# Autodesk Inventor assembly: ASY PRS DrainSystemBottom_940
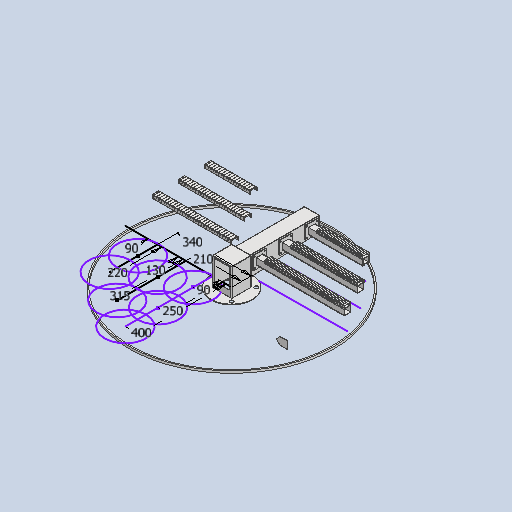
[picture p0: Inventor's stored thumbnail of the model, 512x512]
Saved by Autodesk Inventor 2026.2 (Build 302298000, 298)
## iProperties
Created: 2026-05-12
Part Number: ASY PRS DrainSystemBottom_940
Document SubType Name: Assembly
Designer: admin
Author: admin
## Documents named in this file (20)
- C:\Users\admin\Documents\Inventor\PRS-Purovsk\ASY-PRS-DRS 940.iam
- C:\Users\admin\Documents\Inventor\PRS-Purovsk\PRS-1425 FDS Way FLANGE.ipt
- C:\Users\admin\Documents\Inventor\PRS-Purovsk\ANP 1401 DSB DIMentions.ipt
- C:\Users\admin\Documents\Inventor\PRS-Purovsk\PRS-1662 FDS 1000 way tube 4.ipt
- C:\Users\admin\Documents\Inventor\PRS-Purovsk\PRS-1651 FDS MAIN  FLANGE.ipt
- C:\Users\admin\Documents\Inventor\PRS-Purovsk\PRS-1652 FDS Central tube wall.ipt
- C:\Users\admin\Documents\Inventor\PRS-Purovsk\PRS-1661 FDS 1000 way tube 1.ipt
- C:\Users\admin\Documents\Inventor\PRS-Purovsk\PRS-1662 FDS 1000 way tube 2.ipt
- C:\Users\admin\Documents\Inventor\PRS-Purovsk\PRS-1665 FDS 1000 CUP 1.ipt
- C:\Users\admin\Documents\Inventor\PRS-Purovsk\PRS-1666 FDS 1000 CUP 1.ipt
- C:\Users\admin\Documents\Inventor\PRS-Purovsk\PRS-169859 DIM filter-distribution-system 1000.ipt
- C:\Users\admin\Documents\Inventor\PRS-Purovsk\PRS-1422 BOTTOM FDS diameter way up.ipt
- C:\Users\admin\Documents\Inventor\PRS-Purovsk\PRS-1423 BOTTOM FDS diameter way down.ipt
- C:\Users\admin\Documents\Inventor\PRS-Purovsk\PRS-1424 FDS diam way cup.ipt
- C:\Users\admin\Documents\Inventor\PRS-Purovsk\PRS-531 roof 1.ipt
- C:\Users\admin\Documents\Inventor\PRS-Purovsk\PRS-532 roof 2.ipt
- C:\Users\admin\Documents\Inventor\PRS-Purovsk\PRS-533 roof 3.ipt
- C:\Users\admin\Documents\Inventor\PRS-Purovsk\PRS-531 roof 1940x12.ipt
- C:\Users\admin\Documents\Inventor\PRS-Purovsk\PRS-532 roof 2940x12.ipt
- C:\Users\admin\Documents\Inventor\PRS-Purovsk\PRS-533 roof 3940x12.ipt
## Components (25 placed, 19 different names)
1. PRS-1651 FDS MAIN  FLANGE.ipt:1 — Mate:3, Flush:7, Flush:8
2. PRS-169859 DIM filter-distribution-system 1000.ipt:1 — Mate:1, Mate:2, Flush:1
3. PRS-1425 FDS Way FLANGE.ipt:1 — Rigid:4, Rigid:19
4. ANP 1401 DSB DIMentions.ipt:1
5. PRS-1662 FDS 1000 way tube 4.ipt:1 — Rigid:21, Mate:7, Flush:5, Mate:9
6. PRS-1652 FDS Central tube wall.ipt:1 — Rigid:22, Rigid:24, Flush:7, Flush:8, Mate:10
7. PRS-1652 FDS Central tube wall.ipt:2 — Mate:3, Rigid:22
8. PRS-1662 FDS 1000 way tube 2.ipt:1 — Rigid:20, Mate:6, Flush:6, Mate:8
9. PRS-1665 FDS 1000 CUP 1.ipt:1 — Mate:10
10. PRS-1666 FDS 1000 CUP 1.ipt:1
11. PRS-1422 BOTTOM FDS diameter way up.ipt:1 — Rigid:16, Rigid:17, Rigid:18, Rigid:23, Mate:11, Flush:9, Flush:10
12. PRS-1423 BOTTOM FDS diameter way down.ipt:1 — Rigid:4, Rigid:14, Rigid:15, Rigid:23, Rigid:24
13. PRS-1424 FDS diam way cup.ipt:1 — Mate:11, Flush:9, Flush:10
14. PRS-1425 FDS Way FLANGE.ipt:2 — Rigid:14, Rigid:20
15. PRS-1425 FDS Way FLANGE.ipt:3 — Rigid:15, Rigid:21
16. PRS-1425 FDS Way FLANGE.ipt:4 — Rigid:18
17. PRS-1425 FDS Way FLANGE.ipt:5 — Rigid:17
18. PRS-1425 FDS Way FLANGE.ipt:6 — Rigid:16
19. PRS-1661 FDS 1000 way tube 1.ipt:1 — Rigid:19, Flush:4, Mate:4, Mate:5
20. PRS-531 roof 1:1 — Flush:4, Mate:4, Mate:5
21. PRS-532 roof 2:1 — Mate:6, Flush:6, Mate:8
22. PRS-533 roof 3:1 — Mate:7, Flush:5, Mate:9
23. PRS-531 roof 1940x12:1
24. PRS-532 roof 2940x12:1
25. PRS-533 roof 3940x12:1
## Relationships (31: WeldJoint 12, Mate 11, Flush 8)
- Mate:1: PRS-169859 DIM filter-distribution-system 1000.ipt:1
- Mate:2: PRS-169859 DIM filter-distribution-system 1000.ipt:1
- Flush:1: PRS-169859 DIM filter-distribution-system 1000.ipt:1
- Rigid:4 [WeldJoint]: PRS-1425 FDS Way FLANGE.ipt:1 ↔ PRS-1423 BOTTOM FDS diameter way down.ipt:1
- Mate:3: PRS-1651 FDS MAIN  FLANGE.ipt:1 ↔ PRS-1652 FDS Central tube wall.ipt:2
- Rigid:14 [WeldJoint]: PRS-1423 BOTTOM FDS diameter way down.ipt:1 ↔ PRS-1425 FDS Way FLANGE.ipt:2
- Rigid:15 [WeldJoint]: PRS-1423 BOTTOM FDS diameter way down.ipt:1 ↔ PRS-1425 FDS Way FLANGE.ipt:3
- Rigid:16 [WeldJoint]: PRS-1422 BOTTOM FDS diameter way up.ipt:1 ↔ PRS-1425 FDS Way FLANGE.ipt:6
- Rigid:17 [WeldJoint]: PRS-1422 BOTTOM FDS diameter way up.ipt:1 ↔ PRS-1425 FDS Way FLANGE.ipt:5
- Rigid:18 [WeldJoint]: PRS-1422 BOTTOM FDS diameter way up.ipt:1 ↔ PRS-1425 FDS Way FLANGE.ipt:4
- Rigid:19 [WeldJoint] (-2 mm): PRS-1425 FDS Way FLANGE.ipt:1 ↔ PRS-1661 FDS 1000 way tube 1.ipt:1
- Rigid:20 [WeldJoint] (-2 mm): PRS-1662 FDS 1000 way tube 2.ipt:1 ↔ PRS-1425 FDS Way FLANGE.ipt:2
- Rigid:21 [WeldJoint] (-2 mm): PRS-1662 FDS 1000 way tube 4.ipt:1 ↔ PRS-1425 FDS Way FLANGE.ipt:3
- Rigid:22 [WeldJoint]: PRS-1652 FDS Central tube wall.ipt:1 ↔ PRS-1652 FDS Central tube wall.ipt:2
- Rigid:23 [WeldJoint]: PRS-1422 BOTTOM FDS diameter way up.ipt:1 ↔ PRS-1423 BOTTOM FDS diameter way down.ipt:1
- Rigid:24 [WeldJoint]: PRS-1652 FDS Central tube wall.ipt:1 ↔ PRS-1423 BOTTOM FDS diameter way down.ipt:1
- Flush:4 (40 mm): PRS-1661 FDS 1000 way tube 1.ipt:1 ↔ PRS-531 roof 1:1
- Mate:4: PRS-1661 FDS 1000 way tube 1.ipt:1 ↔ PRS-531 roof 1:1
- Mate:5 (10 mm): PRS-1661 FDS 1000 way tube 1.ipt:1 ↔ PRS-531 roof 1:1
- Mate:6 (10 mm): PRS-1662 FDS 1000 way tube 2.ipt:1 ↔ PRS-532 roof 2:1
- Mate:7 (10 mm): PRS-1662 FDS 1000 way tube 4.ipt:1 ↔ PRS-533 roof 3:1
- Flush:5 (-40 mm): PRS-1662 FDS 1000 way tube 4.ipt:1 ↔ PRS-533 roof 3:1
- Flush:6 (-40 mm): PRS-1662 FDS 1000 way tube 2.ipt:1 ↔ PRS-532 roof 2:1
- Mate:8: PRS-1662 FDS 1000 way tube 2.ipt:1 ↔ PRS-532 roof 2:1
- Mate:9: PRS-1662 FDS 1000 way tube 4.ipt:1 ↔ PRS-533 roof 3:1
- Flush:7: PRS-1651 FDS MAIN  FLANGE.ipt:1 ↔ PRS-1652 FDS Central tube wall.ipt:1
- Flush:8: PRS-1651 FDS MAIN  FLANGE.ipt:1 ↔ PRS-1652 FDS Central tube wall.ipt:1
- Mate:10: PRS-1652 FDS Central tube wall.ipt:1 ↔ PRS-1665 FDS 1000 CUP 1.ipt:1
- Mate:11: PRS-1422 BOTTOM FDS diameter way up.ipt:1 ↔ PRS-1424 FDS diam way cup.ipt:1
- Flush:9 (-1 mm): PRS-1422 BOTTOM FDS diameter way up.ipt:1 ↔ PRS-1424 FDS diam way cup.ipt:1
- Flush:10 (1 mm): PRS-1422 BOTTOM FDS diameter way up.ipt:1 ↔ PRS-1424 FDS diam way cup.ipt:1
